# Autodesk Inventor assembly: MontagemREV0
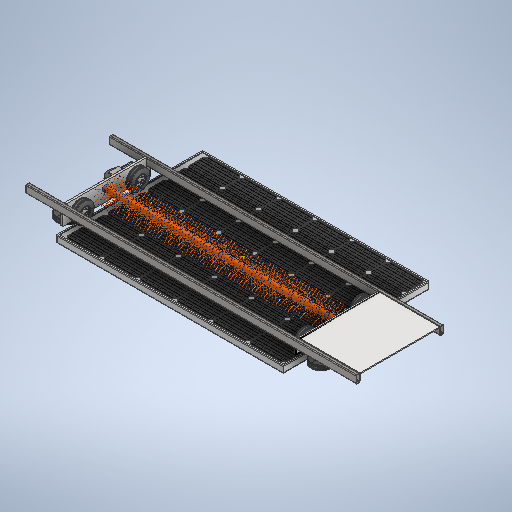
[picture p0: Inventor's stored thumbnail of the model, 512x512]
Saved by Autodesk Inventor 2026.1 (Build 301233020, 233B)
## iProperties
Created: 2025-11-04
Part Number: MontagemREV0
Document SubType Name: Assembly
Designer: Rubens
Author: Rubens
## Documents named in this file (10)
- C:\Users\062210040\Downloads\Limpador Rev2\Limpador reduzido\Limpador reduzido\Limpador\MontagemREV0 - Copia.iam
- C:\Users\062210040\Downloads\Limpador Rev2\Limpador reduzido\Limpador reduzido\Limpador\TCC\aaaaaISO 10799-2 - 40x20x2 - 2600.ipt
- C:\Users\062210040\Downloads\Limpador Rev2\Limpador reduzido\Limpador reduzido\Limpador\TCC\aaaaaPart2.ipt
- C:\Users\062210040\Downloads\Limpador Rev2\Limpador reduzido\Limpador reduzido\Limpador\Teste Suporte.ipt
- C:\Users\062210040\Downloads\Painel reduzido\solar-panel-122.snapshot.3\PV ST SOLAR.ipt
- C:\Users\062210040\Downloads\Limpador Rev2\Limpador reduzido\Limpador reduzido\Limpador\TCC\22874-100-g-a_MIR.ipt
- C:\Users\062210040\Downloads\Limpador Rev2\Limpador reduzido\Limpador reduzido\Limpador\TCC\Suporte Painel1.ipt
- C:\Users\062210040\Downloads\Limpador Rev2\Limpador reduzido\Limpador reduzido\Limpador\TCC\aaaaa22874-100-g-a_MIR.ipt
- C:\Users\062210040\Downloads\sUPORTE1.ipt
- C:\Users\062210040\Downloads\Limpador Rev2\Limpador reduzido\Limpador reduzido\Limpador\EscovãoInicial.ipt
## Components (20 placed, 9 different names)
1. PV ST SOLAR:1 — Flush:2
2. Teste Suporte:3 — Mate:21
3. Teste Suporte:4 — Mate:20
4. 22874-100-g-a_MIR:1 — Mate:16
5. 22874-100-g-a_MIR:2 — Mate:17
6. aaaaaISO 10799-2 - 40x20x2 - 2600:1 — Mate:1, Mate:2, Mate:3, Mate:5
7. aaaaaISO 10799-2 - 40x20x2 - 2600:2 — Mate:1, Mate:2, Mate:4, Flush:1, Mate:6, Mate:22, Mate:23
8. Suporte Painel1:1 — Mate:3, Mate:4, Flush:1, Mate:7
9. aaaaaPart2:2 — Mate:5, Mate:6, Mate:7, Flush:2, Mate:12, Mate:13, Mate:15, Mate:16, Mate:17, Mate:25
10. Teste Suporte:7 — Mate:12, Mate:14, Mate:15
11. Teste Suporte:8 — Mate:13
12. aaaaa22874-100-g-a_MIR:1 — Mate:14
13. aaaaa22874-100-g-a_MIR:2
14. aaaaa22874-100-g-a_MIR:3 — Mate:21
15. aaaaa22874-100-g-a_MIR:4 — Mate:20
16. 22874-100-g-a_MIR:3
17. 22874-100-g-a_MIR:4
18. sUPORTE1:1 — Mate:22, Mate:23
19. EscovãoInicial:1 — Mate:24
20. EscovãoInicial:2 — Mate:24, Mate:25
## Relationships (21: Mate 19, Flush 2)
- Mate:1: aaaaaISO 10799-2 - 40x20x2 - 2600:1 ↔ aaaaaISO 10799-2 - 40x20x2 - 2600:2
- Mate:2 (400 mm): aaaaaISO 10799-2 - 40x20x2 - 2600:1 ↔ aaaaaISO 10799-2 - 40x20x2 - 2600:2
- Mate:3: aaaaaISO 10799-2 - 40x20x2 - 2600:1 ↔ Suporte Painel1:1
- Mate:4: aaaaaISO 10799-2 - 40x20x2 - 2600:2 ↔ Suporte Painel1:1
- Flush:1: aaaaaISO 10799-2 - 40x20x2 - 2600:2 ↔ Suporte Painel1:1
- Mate:5: aaaaaISO 10799-2 - 40x20x2 - 2600:1 ↔ aaaaaPart2:2
- Mate:6: aaaaaISO 10799-2 - 40x20x2 - 2600:2 ↔ aaaaaPart2:2
- Mate:7: Suporte Painel1:1 ↔ aaaaaPart2:2
- Flush:2 (75 mm): PV ST SOLAR:1 ↔ aaaaaPart2:2
- Mate:12: aaaaaPart2:2 ↔ Teste Suporte:7
- Mate:13: aaaaaPart2:2 ↔ Teste Suporte:8
- Mate:14: Teste Suporte:7 ↔ aaaaa22874-100-g-a_MIR:1
- Mate:15: aaaaaPart2:2 ↔ Teste Suporte:7
- Mate:16: 22874-100-g-a_MIR:1 ↔ aaaaaPart2:2
- Mate:17: 22874-100-g-a_MIR:2 ↔ aaaaaPart2:2
- Mate:20: Teste Suporte:4 ↔ aaaaa22874-100-g-a_MIR:4
- Mate:21: Teste Suporte:3 ↔ aaaaa22874-100-g-a_MIR:3
- Mate:22: aaaaaISO 10799-2 - 40x20x2 - 2600:2 ↔ sUPORTE1:1
- Mate:23: aaaaaISO 10799-2 - 40x20x2 - 2600:2 ↔ sUPORTE1:1
- Mate:24: EscovãoInicial:1 ↔ EscovãoInicial:2
- Mate:25: aaaaaPart2:2 ↔ EscovãoInicial:2
